# Autodesk Inventor assembly: Cabina
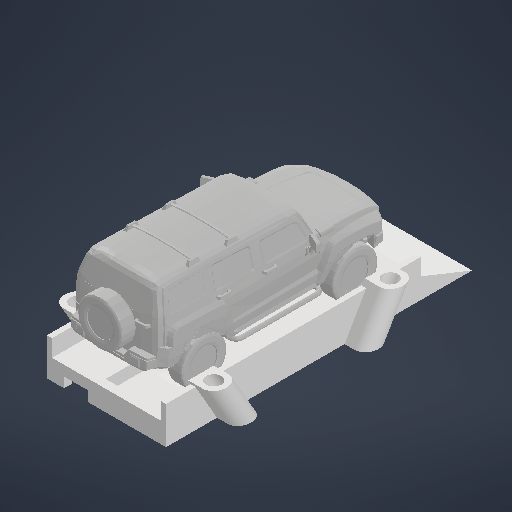
[picture p0: Inventor's stored thumbnail of the model, 512x512]
Saved by Autodesk Inventor 2026.1 (Build 301233020, 233B)
## iProperties
Created: 2025-10-16
Part Number: Cabina
Document SubType Name: Assembly
Designer: tito.luyo
Author: tito.luyo
## Documents named in this file (3)
- C:\work\verticalparking\diseno3d\01_Partes\Cabina.iam
- C:\work\verticalparking\diseno3d\01_Partes\BaseCabina.ipt
- C:\work\verticalparking\diseno3d\01_Partes\external\hammer_h3_v2\HermesH3v2.ipt
## Components (2 placed, 2 different names)
1. BaseCabina:1 — Mate:1
2. HermesH3v2:1 — Mate:1
## Relationships (1: Mate 1)
- Mate:1: BaseCabina:1 ↔ HermesH3v2:1
